# Autodesk Inventor assembly: Molde Base 1
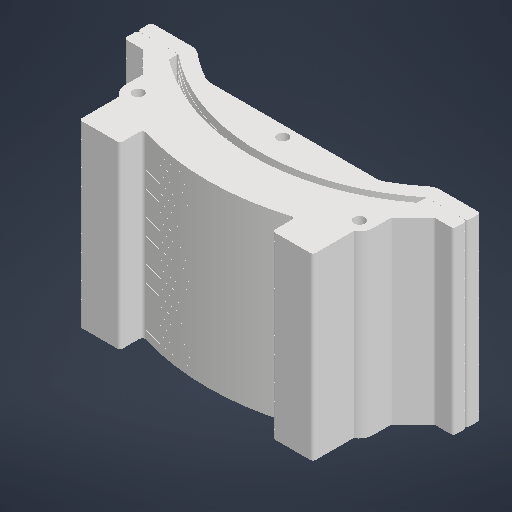
[picture p0: Inventor's stored thumbnail of the model, 512x512]
Saved by Autodesk Inventor 2026.2 (Build 302298000, 298)
## iProperties
Created: 2026-02-26
Part Number: Molde Base 1
Document SubType Name: Assembly
Designer: 06aar
Author: 06aar
## Documents named in this file (4)
- C:\Users\06aar\Documents\GitHub\Atta-Bot-STEM-Fork-aavalerin\Chasis\Diseño V3.0\Molde para Curva Trasera\Molde Base 1.iam
- C:\Users\06aar\Documents\GitHub\Atta-Bot-STEM-Fork-aavalerin\Chasis\Diseño V3.0\Molde para Curva Trasera\Parte A Dos piezas.ipt
- C:\Users\06aar\Documents\GitHub\Atta-Bot-STEM-Fork-aavalerin\Chasis\Diseño V3.0\Molde para Curva Trasera\Parte B bastantes piezas.ipt
- C:\Users\06aar\Documents\GitHub\Atta-Bot-STEM-Fork-aavalerin\Chasis\Diseño V3.0\Molde para Curva Trasera\Pieza Contramolde.ipt
## Components (44 placed, 3 different names)
1. Parte A Dos piezas:1 — Mate:1, Mate:2, Flush:1, Flush:3, Mate:5
2. Parte A Dos piezas:2 — Mate:1, Mate:2, Flush:1, Mate:3, Mate:4, Flush:2
3. Parte B bastantes piezas:1 — Mate:3, Mate:4, Flush:2
4. Parte B bastantes piezas:2
5. Parte B bastantes piezas:3
6. Parte B bastantes piezas:4
7. Parte B bastantes piezas:5
8. Parte B bastantes piezas:6
9. Parte B bastantes piezas:7
10. Parte B bastantes piezas:8
11. Parte B bastantes piezas:9
12. Parte B bastantes piezas:10
13. Parte B bastantes piezas:11
14. Parte B bastantes piezas:12
15. Parte B bastantes piezas:13
16. Parte B bastantes piezas:14
17. Parte B bastantes piezas:15
18. Parte B bastantes piezas:16
19. Parte B bastantes piezas:17
20. Parte B bastantes piezas:18
21. Parte B bastantes piezas:19
22. Parte B bastantes piezas:20
23. Pieza Contramolde:1 — Flush:3, Mate:5
24. Pieza Contramolde:2
25. Pieza Contramolde:3
26. Pieza Contramolde:4
27. Pieza Contramolde:5
28. Pieza Contramolde:6
29. Pieza Contramolde:7
30. Pieza Contramolde:8
31. Pieza Contramolde:9
32. Pieza Contramolde:10
33. Pieza Contramolde:11
34. Pieza Contramolde:12
35. Pieza Contramolde:13
36. Pieza Contramolde:14
37. Pieza Contramolde:15
38. Pieza Contramolde:16
39. Pieza Contramolde:17
40. Pieza Contramolde:18
41. Pieza Contramolde:19
42. Pieza Contramolde:20
43. Pieza Contramolde:21
44. Pieza Contramolde:22
## Component patterns: (20 elements, first: Parte B bastantes piezas:1), (22 elements, first: Pieza Contramolde:1)
## Relationships (8: Mate 5, Flush 3)
- Mate:1: Parte A Dos piezas:1 ↔ Parte A Dos piezas:2
- Mate:2: Parte A Dos piezas:1 ↔ Parte A Dos piezas:2
- Flush:1: Parte A Dos piezas:1 ↔ Parte A Dos piezas:2
- Mate:3: Parte A Dos piezas:2 ↔ Parte B bastantes piezas:1
- Mate:4: Parte A Dos piezas:2 ↔ Parte B bastantes piezas:1
- Flush:2: Parte A Dos piezas:2 ↔ Parte B bastantes piezas:1
- Flush:3: Parte A Dos piezas:1 ↔ Pieza Contramolde:1
- Mate:5: Parte A Dos piezas:1 ↔ Pieza Contramolde:1
